# Autodesk Inventor assembly: FEM-Träger-Baugruppe1
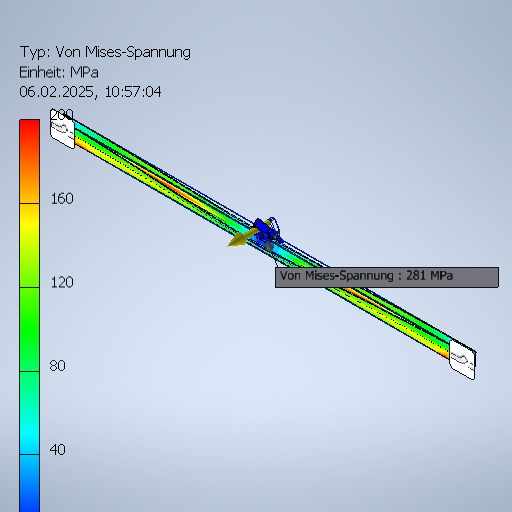
[picture p0: Inventor's stored thumbnail of the model, 512x512]
Saved by Autodesk Inventor 2025 (Build 290162010, 162A)
## iProperties
Created: 2025-02-02
Part Number: FEM-Träger-Baugruppe1
Document SubType Name: Assembly
Designer: Admin
Mass: 451.767 g
Surface Area: 1812.74 cm^2
Volume: 169.619 cm^3
Density: 2.66341 g/cm^3
Author: Admin
## Documents named in this file (10)
- C:\Users\Admin\GIT\HDVKBM\CAD\Krandemonstrator\FEM-Träger-Baugruppe3.iam
- C:\Users\Admin\GIT\HDVKBM\CAD\Krandemonstrator\Träger.ipt
- C:\Users\Admin\GIT\HDVKBM\CAD\Krandemonstrator\Einspannungsfläche.ipt
- C:\Users\Admin\GIT\HDVKBM\CAD\Krandemonstrator\KatzeFEM.iam
- C:\Users\Admin\GIT\HDVKBM\CAD\Krandemonstrator\FEM-Träger-Baugruppe3\AIP\FEA\eym8wc95s.fins
- C:\Users\Admin\GIT\HDVKBM\CAD\Krandemonstrator\FEM-Träger-Baugruppe3\AIP\FEA\eym8wc95s.fsat
- C:\Users\Admin\GIT\HDVKBM\CAD\Krandemonstrator\FEM-Träger-Baugruppe3\AIP\FEA\eym8wc95s.ftes
- C:\Users\Admin\GIT\HDVKBM\CAD\Krandemonstrator\FEM-Träger-Baugruppe3\AIP\FEA\eym8wc95s.fwiz
- C:\Users\Admin\GIT\HDVKBM\CAD\Krandemonstrator\FEM-Träger-Baugruppe3\AIP\FEA\eym8wc97k.fmsh
- C:\Users\Admin\GIT\HDVKBM\CAD\Krandemonstrator\FEM-Träger-Baugruppe3\AIP\FEA\eym8wc97l.fres
## Components (4 placed, 3 different names)
1. Träger:1 — Starr:1, Starr:2, Verschiebbar:4
2. Einspannungsfläche:1 — Starr:1
3. Einspannungsfläche:2 — Starr:2
4. KatzeFEM:1 [sub-assembly] — Verschiebbar:4
## Relationships (3: WeldJoint 2, TranslationJoint 1)
- Starr:1 [WeldJoint]: Träger:1 ↔ Einspannungsfläche:1
- Starr:2 [WeldJoint]: Träger:1 ↔ Einspannungsfläche:2
- Verschiebbar:4 [TranslationJoint] (0.1 mm): Träger:1 ↔ KatzeFEM:1
## Named parameters: sa_0 = 50000
note: some values were not read from the file. Shown as the stored number, unit unknown: "sa_0".
